# Autodesk Inventor assembly: ForeArmAssembly
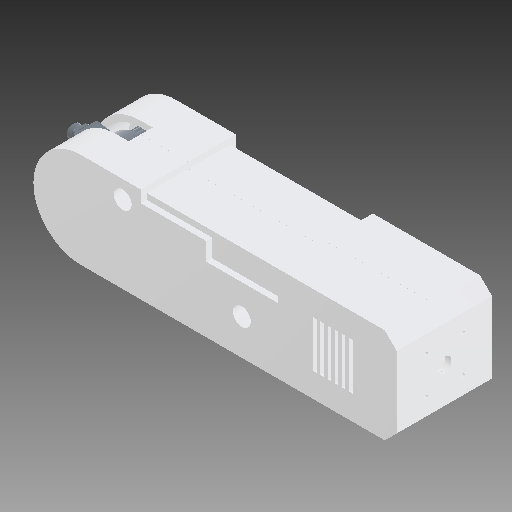
[picture p0: Inventor's stored thumbnail of the model, 512x512]
Saved by Autodesk Inventor 2017 SP1 (Build 210196100, 196)
## iProperties
Created: 2017-06-16
Part Number: ForeArmAssembly
Document SubType Name: Assembly
Designer: Zach
Author: Zach
## Documents named in this file (14)
- C:\Users\Zach\Documents\GitHub\cr-laundry-robot\src\Body\Arm Assembly\Fore Arm Assembly\ForeArmAssembly.iam
- C:\Users\Zach\Documents\GitHub\cr-laundry-robot\src\Body\Arm Assembly\Fore Arm Assembly\FA001.ipt
- C:\Users\Zach\Documents\GitHub\cr-laundry-robot\src\Body\Arm Assembly\Fore Arm Assembly\FA002.ipt
- C:\Users\Zach\Documents\GitHub\cr-laundry-robot\src\Body\Arm Assembly\Fore Arm Assembly\FA003.ipt
- C:\Users\Zach\Documents\GitHub\cr-laundry-robot\src\Body\Arm Assembly\Fore Arm Assembly\FA004.ipt
- C:\Users\Zach\Documents\GitHub\cr-laundry-robot\src\Body\Arm Assembly\Fore Arm Assembly\FA005.ipt
- C:\Users\Zach\Documents\GitHub\cr-laundry-robot\lib\Stepper Motor - NEMA 17\NEMA17.ipt
- C:\Users\Zach\Documents\GitHub\cr-laundry-robot\src\Body\Arm Assembly\Fore Arm Assembly\FA006.ipt
- C:\Users\Zach\Documents\GitHub\cr-laundry-robot\src\Body\Arm Assembly\Fore Arm Assembly\FA007.ipt
- C:\Users\Zach\Documents\GitHub\cr-laundry-robot\src\Body\Arm Assembly\Fore Arm Assembly\FA008.ipt
- C:\Users\Zach\Documents\GitHub\cr-laundry-robot\lib\Futaba S3114\FutabaS3114.ipt
- C:\Users\Zach\Documents\GitHub\cr-laundry-robot\src\Body\Arm Assembly\Fore Arm Assembly\FA009.ipt
- C:\Users\Zach\Documents\GitHub\cr-laundry-robot\src\Body\Arm Assembly\Fore Arm Assembly\FA010.ipt
- C:\Users\Zach\Documents\GitHub\cr-laundry-robot\src\Body\Arm Assembly\Fore Arm Assembly\FA011.ipt
## Components (14 placed, 13 different names)
1. FA001:1 — Mate:3, Mate:4, Mate:12, Mate:13, Mate:14, Mate:15, Mate:16
2. FA002:1 — Mate:15, Mate:16
3. FA003:1 — Mate:3, Mate:4, Mate:10, Mate:11, Mate:20, Mate:21, Mate:28, Mate:29, Mate:30, Mate:34
4. FA004:1 — Mate:40, Mate:42, Mate:43, Mate:44
5. FA005:1 — Mate:10, Mate:11, Mate:25, Mate:35, Mate:36, Mate:38
6. NEMA17:1 — Mate:12, Mate:13, Mate:14
7. NEMA17:2 — Mate:22, Mate:28, Mate:29, Mate:30
8. FA006:1 — Mate:20, Mate:21, Mate:42, Mate:43
9. FA007:1 — Mate:22, Mate:34, Rotation:2
10. FA008:1 — Mate:25, Mate:31, Mate:32, Mate:33, Mate:39, Mate:41, Rotation:3
11. FutabaS3114:1 — Mate:31, Mate:32, Mate:33
12. FA009:1 — Mate:35, Mate:36, Mate:37
13. FA010:1 — Mate:37, Mate:38, Rotation:2, Rotation:3
14. FA011:1 — Mate:39, Mate:40, Mate:41, Mate:44
## Relationships (32: Mate 30, RelateRotation 2)
- Mate:3: FA001:1 ↔ FA003:1
- Mate:4: FA001:1 ↔ FA003:1
- Mate:10: FA003:1 ↔ FA005:1
- Mate:11: FA003:1 ↔ FA005:1
- Mate:12: FA001:1 ↔ NEMA17:1
- Mate:13: FA001:1 ↔ NEMA17:1
- Mate:14: FA001:1 ↔ NEMA17:1
- Mate:15: FA001:1 ↔ FA002:1
- Mate:16: FA001:1 ↔ FA002:1
- Mate:20: FA003:1 ↔ FA006:1
- Mate:21: FA003:1 ↔ FA006:1
- Mate:22: NEMA17:2 ↔ FA007:1
- Mate:25: FA005:1 ↔ FA008:1
- Mate:28: FA003:1 ↔ NEMA17:2
- Mate:29: FA003:1 ↔ NEMA17:2
- Mate:30: FA003:1 ↔ NEMA17:2
- Mate:31: FA008:1 ↔ FutabaS3114:1
- Mate:32: FA008:1 ↔ FutabaS3114:1
- Mate:33: FA008:1 ↔ FutabaS3114:1
- Mate:34: FA003:1 ↔ FA007:1
- Mate:35: FA005:1 ↔ FA009:1
- Mate:36: FA005:1 ↔ FA009:1
- Mate:37: FA009:1 ↔ FA010:1
- Mate:38: FA005:1 ↔ FA010:1
- Rotation:2 [RelateRotation] (0.7778 ul): FA007:1 ↔ FA010:1
- Mate:39: FA008:1 ↔ FA011:1
- Mate:40: FA004:1 ↔ FA011:1
- Mate:41: FA008:1 ↔ FA011:1
- Rotation:3 [RelateRotation] (0.5 ul): FA008:1 ↔ FA010:1
- Mate:42: FA004:1 ↔ FA006:1
- Mate:43: FA004:1 ↔ FA006:1
- Mate:44: FA004:1 ↔ FA011:1
